# Autodesk Inventor assembly: SM_ZA01
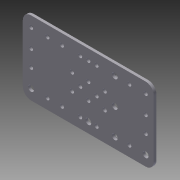
[picture p0: Inventor's stored thumbnail of the model, 180x180]
Saved by Autodesk Inventor 2013 (Build 170138000, 138)
## iProperties
Created: 2012-05-01
Part Number: SM_ZA01
Document SubType Name: Assembly
Designer: ERF
Stock Number: SM_ZA01
Author: ERF
Title: Z Axis Mount Plate Assembly
## Documents named in this file (3)
- C:\Users\Brett\Documents\GitHub\BigOko\Assemblies\SM-ZA01.iam
- C:\Users\Brett\Documents\GitHub\BigOko\Parts\MSK01-01.ipt
- C:\Users\Brett\Documents\GitHub\BigOko\Parts\SM-H03.ipt
## Components (5 placed, 2 different names)
1. MSK01-01:1 — Insert:4, Insert:5, Mate:2, Mate:4
2. SM-H03:1 — Mate:4
3. SM-H03:2 — Mate:2
4. SM-H03:3 — Insert:5
5. SM-H03:4 — Insert:4
## Relationships (4: Insert 2, Mate 2)
- Insert:4: MSK01-01:1 ↔ SM-H03:4
- Insert:5: MSK01-01:1 ↔ SM-H03:3
- Mate:2: MSK01-01:1 ↔ SM-H03:2
- Mate:4: MSK01-01:1 ↔ SM-H03:1
